# Autodesk Inventor assembly: Shooter Oct14
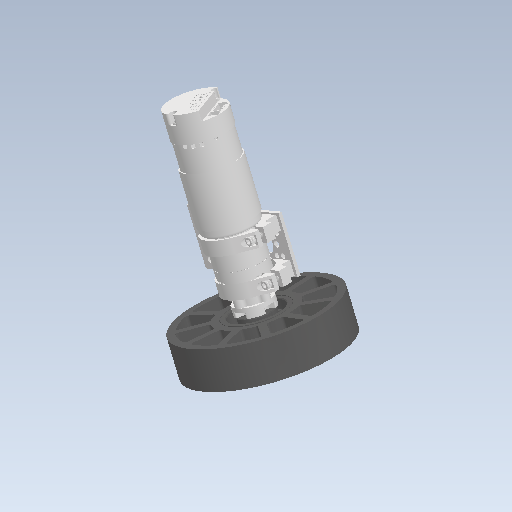
[picture p0: Inventor's stored thumbnail of the model, 512x512]
Saved by Autodesk Inventor 2020.3 (Build 243373000, 373)
## iProperties
Created: 2020-10-14
Part Number: Shooter Oct14
Document SubType Name: Assembly
Designer: Owner
Author: Owner
## Documents named in this file (7)
- C:\Users\19713\Documents\GitHub\CAD-2021-Ultimate_Goal\Shooter\ShooterNoBoard.iam
- C:\Users\19713\Documents\GitHub\CAD-2021-Ultimate_Goal\GoBilda\5202-0002-0003 part.ipt
- C:\Users\19713\Documents\GitHub\CAD-2021-Ultimate_Goal\ServoCity\555176 assembly.ipt
- C:\Users\19713\Documents\GitHub\CAD-2021-Ultimate_Goal\AndyMark\am-3563 4IN 8mm Round Compliant Wheel REV2.ipt
- C:\Users\19713\Documents\GitHub\CAD-2021-Ultimate_Goal\ServoCity\545456.ipt
- C:\Users\19713\Documents\GitHub\CAD-2021-Ultimate_Goal\ServoCity\545636 assembly.ipt
- C:\Users\19713\Documents\GitHub\CAD-2021-Ultimate_Goal\ServoCity\585720.ipt
## Components (7 placed, 6 different names)
1. 5202-0002-0003 part:1 — Mate:20, Mate:22, Mate:29, Mate:30
2. 555176 assembly:1 — Mate:23, Mate:24, Mate:27, Mate:28, Mate:29, Mate:30
3. 555176 assembly:2 — Mate:25, Mate:26
4. am-3563 4IN 8mm Round Compliant Wheel REV2:1 — Mate:19
5. 545456:1 — Mate:19
6. 545636 assembly:1 — Mate:20, Mate:22
7. 585720:1 — Mate:23, Mate:24, Mate:25, Mate:26, Mate:27, Mate:28
## Relationships (16: Mate 16)
- [Mate]: 545456:1 ↔ 545636 assembly:1
- [Mate]: 545456:1 ↔ 545636 assembly:1
- [Mate]: 545456:1 ↔ 545636 assembly:1
- [Mate]: am-3563 4IN 8mm Round Compliant Wheel REV2:1 ↔ 545456:1
- [Mate]: am-3563 4IN 8mm Round Compliant Wheel REV2:1 ↔ 545456:1
- Mate:19: am-3563 4IN 8mm Round Compliant Wheel REV2:1 ↔ 545456:1
- Mate:20: 5202-0002-0003 part:1 ↔ 545636 assembly:1
- Mate:22: 5202-0002-0003 part:1 ↔ 545636 assembly:1
- Mate:23: 555176 assembly:1 ↔ 585720:1
- Mate:24: 555176 assembly:1 ↔ 585720:1
- Mate:25: 555176 assembly:2 ↔ 585720:1
- Mate:26: 555176 assembly:2 ↔ 585720:1
- Mate:27: 555176 assembly:1 ↔ 585720:1
- Mate:28: 555176 assembly:1 ↔ 585720:1
- Mate:29: 5202-0002-0003 part:1 ↔ 555176 assembly:1
- Mate:30: 5202-0002-0003 part:1 ↔ 555176 assembly:1
## Named parameters: d13_d14 = 0 mm, d14_d17 = 0 mm
